# Autodesk Inventor assembly: Front Left Wheel Hub Assemby
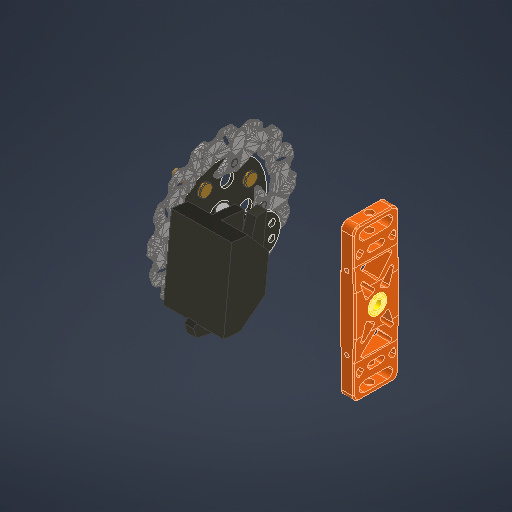
[picture p0: Inventor's stored thumbnail of the model, 512x512]
Saved by Autodesk Inventor 2026.1 (Build 301233000, 233)
## iProperties
Created: 2026-06-24
Part Number: Front Left Wheel Hub Assemby
Document SubType Name: Assembly
Designer: share
Author: share
## Documents named in this file (6)
- C:\Users\share\OneDrive\Documents\Personal Projects\GOGO Kart\CAD\GOGO_KART_FSAE\Suspension\Upright Assembly\Front Left Wheel Hub Assemby.iam
- C:\Users\share\OneDrive\Documents\Personal Projects\GOGO Kart\CAD\GOGO_KART_FSAE\Suspension\Upright Assembly\Front Upright.ipt
- C:\Users\share\OneDrive\Documents\Personal Projects\GOGO Kart\CAD\GOGO_KART_FSAE\Suspension\Upright Assembly\F3 Front Caliper Bracket.ipt
- C:\Users\share\OneDrive\Documents\Personal Projects\GOGO Kart\CAD\GOGO_KART_FSAE\Drivetrain\Rear_Wheel_Hub_Assembly.iam
- C:\Users\share\OneDrive\Documents\Personal Projects\GOGO Kart\CAD\GOGO_KART_FSAE\Suspension\Upright Assembly\Arashi Rear Brake Disc Rotors.ipt
- C:\Users\share\Downloads\2385K101_Angular Contact Single Row Ball Bearing\2385K101_Angular Contact Single Row Ball Bearing\2385K101_Angular Contact Single Row Ball Bearing.ipt
## Components (6 placed, 5 different names)
1. Front Upright:1 — Flush:1, Flush:2, Flush:3, Mate:1, Insert:5, Insert:6
2. F3 Front Caliper Bracket:1
3. Rear_Wheel_Hub_Assembly:1 [sub-assembly] — Mate:1, Insert:3, Insert:4
4. Arashi Rear Brake Disc Rotors:1 — Insert:3, Insert:4
5. 2385K101_Angular Contact Single Row Ball Bearing:1 — Insert:6
6. 2385K101_Angular Contact Single Row Ball Bearing:2 — Insert:5
## Relationships (8: Insert 4, Flush 3, Mate 1)
- Flush:1: Front Upright:1
- Flush:2: Front Upright:1
- Flush:3: Front Upright:1
- Mate:1: Front Upright:1 ↔ Rear_Wheel_Hub_Assembly:1
- Insert:3: Rear_Wheel_Hub_Assembly:1 ↔ Arashi Rear Brake Disc Rotors:1
- Insert:4: Rear_Wheel_Hub_Assembly:1 ↔ Arashi Rear Brake Disc Rotors:1
- Insert:5: Front Upright:1 ↔ 2385K101_Angular Contact Single Row Ball Bearing:2
- Insert:6: Front Upright:1 ↔ 2385K101_Angular Contact Single Row Ball Bearing:1
